# Autodesk Inventor assembly: 536331 ADN-16-50-A-P-A---(asm_0)
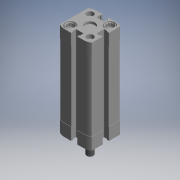
[picture p0: Inventor's stored thumbnail of the model, 180x180]
Saved by Autodesk Inventor 2017.3 (Build 213256000, 256)
## iProperties
Category: PARTsolutions
Company: FESTO
Part Number: 536331 ADN-16-50-A-P-A---(asm_0)
Catalog Web Link: www.cadenas.de
Description: ADN-Compact cylinder
Vendor: FESTO
Document SubType Name: Assembly
Designer: partserver
Manufacturer: FESTO
Mass: 149 g
Surface Area: 255.195 cm^2
Volume: 48.6263 cm^3
Density: 3.06419 g/cm^3
Title: 536331 ADN-16-50-A-P-A
Author: Cadenas PARTsolutions
Comments: Compact cylinder
PSOL_IDENT_0: {ATYP=ASSISTANT},{DATA=script=$CADENAS_DATA/23d-libs/festo/webfesto.vbb/&M_FAMILY=ADN&M_GROUP=01&M_P
PSOL_IDENT_1: ARTNO=536331&IDCODE1=ADN-16-50-A-P-A&IDCODE2=&customer_number_cns=&MATES=1&LOD=HI&LOCKERP=0&SINGLEPA
PSOL_IDENT_2: RT=1}
NB: 536331 ADN-16-50-A-P-A---(asm_0)
NN: ADN
NT: Compact cylinder
NBSYN: $TNR. $TYP.---(asm_$HUBST.)
LINA: 536331 ADN-16-50-A-P-A
CATALOG: Festo
OFFICIAL_STANDARD_NUMBERS: ISO 21287
TNR: 536331
TYP: ADN-16-50-A-P-A
KDM: 16
HUB: 50
HUBST: 0
DF: P
TH: A
A: 12
AF: 10
BG: 17
D1: 9
D5: 6
E: 29
EE: M5
G: 11
KF: M4
KK: M6
L3: 3.5
L12: 3.7
MM: 8
PL: 6
RR: 3.2
RT: M4
SW: 7
T1: 2.1
T4: 1.5
TG: 18
WH: 4.7
ZA: 35
ZB: 39.7
J3: 2.6
RA: 0
RU: 18.6
R1: 9.55
R2: 0.6
CNSMASSEXACT: 0.149
SUPPLIER: FESTO
ARTICLENO: 536331 ADN-16-50-A-P-A---(asm_0)
BOMINFO: 536331 ADN-16-50-A-P-A
CREATOR: CADENAS GmbH
## Documents named in this file (3)
- e:\temp\worker_7\temp\exporttempdir_764_4_Ofl34\format_0\536331 ADN-16-50-A-P-A---(asm_0).iam
- e:\temp\worker_7\temp\exporttempdir_764_4_Ofl34\format_0\536218 ADN-50-P---(Z).ipt
- e:\temp\worker_7\temp\exporttempdir_764_4_Ofl34\format_0\536218 ADN-50-P-A_(KS).ipt
## Components (2 placed, 2 different names)
1. 536218 ADN-50-P---(Z):1 — CYLINDER_XY@1 <-> PISTON_XY@2, CYLINDER_Z@1 <-> PISTON_Z@2, CYLINDER_YZ@1 <-> PISTON_YZ@2
2. 536218 ADN-50-P-A_(KS):1 — CYLINDER_XY@1 <-> PISTON_XY@2, CYLINDER_Z@1 <-> PISTON_Z@2, CYLINDER_YZ@1 <-> PISTON_YZ@2
## Relationships (3: Mate 2, Angle 1)
- CYLINDER_XY@1 <-> PISTON_XY@2 [Mate]: 536218 ADN-50-P---(Z):1 ↔ 536218 ADN-50-P-A_(KS):1
- CYLINDER_Z@1 <-> PISTON_Z@2 [Mate]: 536218 ADN-50-P---(Z):1 ↔ 536218 ADN-50-P-A_(KS):1
- CYLINDER_YZ@1 <-> PISTON_YZ@2 [Angle] (0 deg): 536218 ADN-50-P---(Z):1 ↔ 536218 ADN-50-P-A_(KS):1
